# Autodesk Inventor assembly: all형상
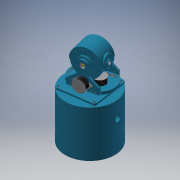
[picture p0: Inventor's stored thumbnail of the model, 180x180]
Saved by Autodesk Inventor 2019 (Build 230136000, 136)
## iProperties
Created: 2018-05-03
Part Number: all형상
Material: 일반
Document SubType Name: Assembly
Designer: CK
Author: CK
## Documents named in this file (3)
- C:\Users\GMIMG\Documents\카카오톡 받은 파일\어셈파일\all형상.iam
- C:\Users\GMIMG\Documents\카카오톡 받은 파일\어셈파일\상부조립.iam
- C:\Users\GMIMG\Documents\카카오톡 받은 파일\어셈파일\바텀조립.iam
## Components (2 placed, 2 different names)
1. 상부조립:1 [sub-assembly] — 메이트:1, 메이트:2, 메이트:3
2. 바텀조립:1 [sub-assembly] — 메이트:1, 메이트:2, 메이트:3, 메이트:4
## Relationships (4: Mate 4)
- 메이트:1 [Mate]: 상부조립:1 ↔ 바텀조립:1
- 메이트:2 [Mate]: 상부조립:1 ↔ 바텀조립:1
- 메이트:3 [Mate]: 상부조립:1 ↔ 바텀조립:1
- 메이트:4 [Mate]: 바텀조립:1
